# Autodesk Inventor assembly: Bush
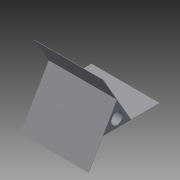
[picture p0: Inventor's stored thumbnail of the model, 180x180]
Saved by Autodesk Inventor 2014 (Build 180170000, 170)
## iProperties
Created: 2014-03-16
Part Number: Bush
Document SubType Name: Assembly
Designer: Pranav
Author: Pranav
## Documents named in this file (3)
- E:\Robotics Autodesk\Bush.iam
- E:\Robotics Autodesk\Triangle.ipt
- E:\Robotics Autodesk\Sweep.ipt
## Components (4 placed, 2 different names)
1. Triangle:1 — Mate:1, Mate:2
2. Sweep:1 — Mate:1, Mate:2
3. Sweep:2
4. Sweep:3
## Component patterns: (3 elements, first: Sweep:1)
## Relationships (2: Mate 2)
- Mate:1: Triangle:1 ↔ Sweep:1
- Mate:2: Triangle:1 ↔ Sweep:1
